# Autodesk Inventor assembly: Assembly2
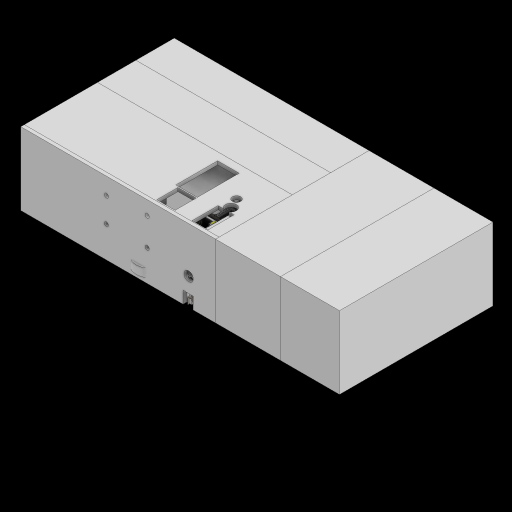
[picture p0: Inventor's stored thumbnail of the model, 512x512]
Saved by Autodesk Inventor 2023 (Build 270158000, 158)
## iProperties
Created: 2022-07-12
Part Number: Assembly2
Document SubType Name: Assembly
Designer: Fuzzyfish
Author: Fuzzyfish
## Documents named in this file (13)
- C:\Users\Fuzzyfish\Documents\Inventor\finalBox\Assembly2.iam
- C:\Users\Fuzzyfish\Documents\Inventor\finalBox\ElecTweetBox.ipt
- C:\Users\Fuzzyfish\Documents\Inventor\finalBox\3waysplitter.ipt
- C:\Users\Fuzzyfish\Documents\Inventor\finalBox\amp.ipt
- C:\Users\Fuzzyfish\Documents\Inventor\finalBox\tweetwe.ipt
- C:\Users\Fuzzyfish\Documents\Inventor\finalBox\acrylicSidePanel.ipt
- C:\Users\Fuzzyfish\Documents\Inventor\finalBox\acrylicBackPanel.ipt
- C:\Users\Fuzzyfish\Documents\Inventor\finalBox\volumeKnob.ipt
- C:\Users\Fuzzyfish\Documents\Inventor\finalBox\midGroove.ipt
- C:\Users\Fuzzyfish\Documents\Inventor\finalBox\midTongue.ipt
- C:\Users\Fuzzyfish\Documents\Inventor\finalBox\rpiWCase.iam
- C:\Users\Fuzzyfish\Documents\Inventor\finalBox\wooferBoxGroove.ipt
- C:\Users\Fuzzyfish\Documents\Inventor\finalBox\wooferBoxTongue.ipt
## Components (12 placed, 12 different names)
1. ElecTweetBox:1 — Flush:4, Flush:5, Flush:6, Mate:30, Mate:31, Mate:32, Mate:33, Mate:34, Mate:39, Mate:40, Flush:9, Mate:41, Flush:11, Flush:14, Mate:44, Flush:15, Mate:45
2. 3waysplitter:1 — Mate:35, Mate:36, Mate:37
3. amp:1 — Mate:13, Mate:14, Mate:15, Flush:4, Flush:5, Mate:47
4. tweetwe:1 — Flush:6, Mate:30, Mate:31
5. acrylicSidePanel:1 — Mate:43, Flush:14, Mate:44, Mate:46
6. acrylicBackPanel:1 — Flush:15, Mate:45, Mate:46
7. volumeKnob:1 — Mate:13, Mate:14, Mate:15
8. midGroove:1 — Mate:42, Flush:12, Flush:13
9. midTongue:1 — Mate:41, Flush:10, Flush:11, Mate:42, Flush:12, Flush:13
10. rpiWCase:1 [sub-assembly] — Mate:32, Mate:33, Mate:34, Mate:47
11. wooferBoxGroove:1 — Flush:7, Flush:8, Mate:35, Mate:36, Mate:37, Mate:38, Mate:39, Mate:40, Flush:9, Flush:10, Mate:43
12. wooferBoxTongue:1 — Flush:7, Flush:8, Mate:38
## Relationships (33: Mate 21, Flush 12)
- Mate:13: amp:1 ↔ volumeKnob:1
- Mate:14: amp:1 ↔ volumeKnob:1
- Mate:15: amp:1 ↔ volumeKnob:1
- Flush:4: ElecTweetBox:1 ↔ amp:1
- Flush:5: ElecTweetBox:1 ↔ amp:1
- Flush:6: ElecTweetBox:1 ↔ tweetwe:1
- Mate:30: ElecTweetBox:1 ↔ tweetwe:1
- Mate:31: ElecTweetBox:1 ↔ tweetwe:1
- Mate:32: ElecTweetBox:1 ↔ rpiWCase:1
- Mate:33 (0.3 mm): ElecTweetBox:1 ↔ rpiWCase:1
- Mate:34 (0.3 mm): ElecTweetBox:1 ↔ rpiWCase:1
- Flush:7: wooferBoxGroove:1 ↔ wooferBoxTongue:1
- Flush:8: wooferBoxGroove:1 ↔ wooferBoxTongue:1
- Mate:35: 3waysplitter:1 ↔ wooferBoxGroove:1
- Mate:36: 3waysplitter:1 ↔ wooferBoxGroove:1
- Mate:37: 3waysplitter:1 ↔ wooferBoxGroove:1
- Mate:38: wooferBoxGroove:1 ↔ wooferBoxTongue:1
- Mate:39: ElecTweetBox:1 ↔ wooferBoxGroove:1
- Mate:40: ElecTweetBox:1 ↔ wooferBoxGroove:1
- Flush:9: ElecTweetBox:1 ↔ wooferBoxGroove:1
- Mate:41: ElecTweetBox:1 ↔ midTongue:1
- Flush:10: midTongue:1 ↔ wooferBoxGroove:1
- Flush:11: ElecTweetBox:1 ↔ midTongue:1
- Mate:42: midGroove:1 ↔ midTongue:1
- Flush:12: midGroove:1 ↔ midTongue:1
- Flush:13: midGroove:1 ↔ midTongue:1
- Mate:43: acrylicSidePanel:1 ↔ wooferBoxGroove:1
- Flush:14: ElecTweetBox:1 ↔ acrylicSidePanel:1
- Mate:44: ElecTweetBox:1 ↔ acrylicSidePanel:1
- Flush:15: ElecTweetBox:1 ↔ acrylicBackPanel:1
- Mate:45: ElecTweetBox:1 ↔ acrylicBackPanel:1
- Mate:46: acrylicSidePanel:1 ↔ acrylicBackPanel:1
- Mate:47 (20 mm): amp:1 ↔ rpiWCase:1
